# Autodesk Inventor assembly: ServoHousingAssembly
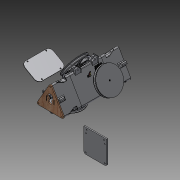
[picture p0: Inventor's stored thumbnail of the model, 180x180]
Saved by Autodesk Inventor 2014 SP1 (Build 180222100, 222)
## iProperties
Created: 2014-11-03
Part Number: ServoHousingAssembly
Document SubType Name: Assembly
Designer: rawrdong
Author: rawrdong
## Documents named in this file (8)
- C:\Users\rawrdong\Documents\GitHub\FlippityFlappity\CAD_HW\ServoHousingAssembly.iam
- C:\Users\rawrdong\Documents\GitHub\FlippityFlappity\CAD_HW\servo-6.snapshot.1\Imported Components\Servo HS425BB\Servo HS425BB.ipt
- C:\Users\rawrdong\Documents\GitHub\FlippityFlappity\CAD_HW\ServoHousingEndPlates.ipt
- C:\Users\rawrdong\Documents\GitHub\FlippityFlappity\CAD_HW\ServoHousing3X.ipt
- C:\Users\rawrdong\Documents\GitHub\FlippityFlappity\CAD_HW\Imported Components\mbed_DanielLim\mbed_DanielLim.ipt
- C:\Users\rawrdong\Documents\GitHub\FlippityFlappity\CAD_HW\MotorSection.ipt
- C:\Users\rawrdong\Documents\GitHub\FlippityFlappity\CAD_HW\Spool.ipt
- C:\Users\rawrdong\Documents\GitHub\FlippityFlappity\CAD_HW\electronics_pouch.ipt
## Components (13 placed, 7 different names)
1. Servo HS425BB:1 — Mate:3, Mate:13, Mate:14, Mate:20
2. Servo HS425BB:2 — Mate:2, Mate:11, Mate:12, Mate:17
3. Servo HS425BB:3 — Mate:1, Mate:16, Mate:18, Mate:19
4. ServoHousingEndPlates:1 — Mate:4, Mate:5, Mate:6
5. ServoHousing3X:2 — Mate:1, Mate:2, Mate:3, Mate:4, Mate:5, Mate:6, Flush:1, Flush:2, Mate:16, Mate:17, Mate:20, Mate:22, Mate:23, Mate:24, Mate:25, Mate:26, Mate:27
6. mbed_DanielLim:1 — Mate:25, Mate:26, Mate:27
7. MotorSection:1 — Flush:1, Flush:2, Mate:8, Mate:9, Mate:10
8. ServoHousingEndPlates:2 — Mate:8, Mate:9, Mate:10
9. Spool:1 — Mate:11, Mate:12
10. Spool:2 — Mate:13, Mate:14
11. Spool:3 — Mate:18, Mate:19
12. MotorSection:2 — Mate:22, Mate:23, Mate:24
13. electronics_pouch:1
## Relationships (26: Mate 24, Flush 2)
- Mate:1: Servo HS425BB:3 ↔ ServoHousing3X:2
- Mate:2: Servo HS425BB:2 ↔ ServoHousing3X:2
- Mate:3: Servo HS425BB:1 ↔ ServoHousing3X:2
- Mate:4: ServoHousingEndPlates:1 ↔ ServoHousing3X:2
- Mate:5: ServoHousingEndPlates:1 ↔ ServoHousing3X:2
- Mate:6: ServoHousingEndPlates:1 ↔ ServoHousing3X:2
- Flush:1: ServoHousing3X:2 ↔ MotorSection:1
- Flush:2: ServoHousing3X:2 ↔ MotorSection:1
- Mate:8: MotorSection:1 ↔ ServoHousingEndPlates:2
- Mate:9: MotorSection:1 ↔ ServoHousingEndPlates:2
- Mate:10: MotorSection:1 ↔ ServoHousingEndPlates:2
- Mate:11: Servo HS425BB:2 ↔ Spool:1
- Mate:12: Servo HS425BB:2 ↔ Spool:1
- Mate:13: Servo HS425BB:1 ↔ Spool:2
- Mate:14: Servo HS425BB:1 ↔ Spool:2
- Mate:16: Servo HS425BB:3 ↔ ServoHousing3X:2
- Mate:17: Servo HS425BB:2 ↔ ServoHousing3X:2
- Mate:18: Servo HS425BB:3 ↔ Spool:3
- Mate:19: Servo HS425BB:3 ↔ Spool:3
- Mate:20: Servo HS425BB:1 ↔ ServoHousing3X:2
- Mate:22: ServoHousing3X:2 ↔ MotorSection:2
- Mate:23: ServoHousing3X:2 ↔ MotorSection:2
- Mate:24: ServoHousing3X:2 ↔ MotorSection:2
- Mate:25: ServoHousing3X:2 ↔ mbed_DanielLim:1
- Mate:26: ServoHousing3X:2 ↔ mbed_DanielLim:1
- Mate:27: ServoHousing3X:2 ↔ mbed_DanielLim:1
